# Autodesk Inventor assembly: Center Wheel
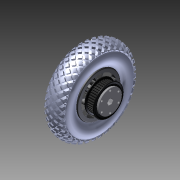
[picture p0: Inventor's stored thumbnail of the model, 180x180]
Saved by Autodesk Inventor 2014 SP1 (Build 180222100, 222)
## iProperties
Created: 2014-01-21
Part Number: Center Wheel
Document SubType Name: Assembly
Designer: Nick
Author: Nick
## Documents named in this file (4)
- D:\Dropbox\School\PurdueFIRST\PFP Robot\PFP Robot with Cart\Center Wheel.iam
- D:\Dropbox\School\PurdueFIRST\PFP Robot\PFP Robot with Cart\PneumaticWheel_am-0970.iam
- D:\Dropbox\School\PurdueFIRST\PFP Robot\PFP Robot with Cart\Pulley.iam
- D:\Dropbox\School\PurdueFIRST\PFP Robot\PFP Robot with Cart\Imported Components\500_hex_hub\500_hex_hub.ipt
## Components (5 placed, 3 different names)
1. PneumaticWheel_am-0970:1 [sub-assembly] — Insert:1, Insert:2, Insert:3, Insert:4
2. Pulley:1 [sub-assembly] — Insert:3, Insert:4, Mate:4, Mate:5, Mate:6
3. Pulley:2 [sub-assembly] — Insert:1, Insert:2, Mate:1, Mate:2, Mate:3
4. 500_hex_hub:1 — Mate:1, Mate:2, Mate:3
5. 500_hex_hub:2 — Mate:4, Mate:5, Mate:6
## Relationships (10: Mate 6, Insert 4)
- Insert:1 (9.525 mm): PneumaticWheel_am-0970:1 ↔ Pulley:2
- Insert:2 (9.525 mm): PneumaticWheel_am-0970:1 ↔ Pulley:2
- Insert:3 (9.525 mm): PneumaticWheel_am-0970:1 ↔ Pulley:1
- Insert:4 (9.525 mm): PneumaticWheel_am-0970:1 ↔ Pulley:1
- Mate:1: Pulley:2 ↔ 500_hex_hub:1
- Mate:2: Pulley:2 ↔ 500_hex_hub:1
- Mate:3: Pulley:2 ↔ 500_hex_hub:1
- Mate:4: Pulley:1 ↔ 500_hex_hub:2
- Mate:5: Pulley:1 ↔ 500_hex_hub:2
- Mate:6: Pulley:1 ↔ 500_hex_hub:2
